# Autodesk Inventor assembly: Shade 02 with LEDs 01
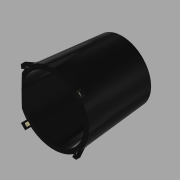
[picture p0: Inventor's stored thumbnail of the model, 180x180]
Saved by Autodesk Inventor 2020 (Build 240168000, 168)
## iProperties
Created: 2019-07-25
Part Number: Shade 02 with LEDs 01
Document SubType Name: Assembly
Designer: Ben
Author: Ben
## Documents named in this file (3)
- C:\Users\Ben\Documents\Inventor\HydraVivarium\Shade 02 with LEDs 01.iam
- C:\Users\Ben\Documents\Inventor\HydraVivarium\Lens Shade and Light 02.ipt
- C:\Users\Ben\Documents\Inventor\HydraVivarium\SFH4451 Narrow Beam IR LED.ipt
## Components (5 placed, 2 different names)
1. Lens Shade and Light 02:1 — Mate:1, Mate:2, Mate:3
2. SFH4451 Narrow Beam IR LED:1 — Mate:1, Mate:2, Mate:3
3. SFH4451 Narrow Beam IR LED:2
4. SFH4451 Narrow Beam IR LED:3
5. SFH4451 Narrow Beam IR LED:4
## Component patterns: (4 elements, first: SFH4451 Narrow Beam IR LED:1)
## Relationships (3: Mate 3)
- Mate:1: Lens Shade and Light 02:1 ↔ SFH4451 Narrow Beam IR LED:1
- Mate:2: Lens Shade and Light 02:1 ↔ SFH4451 Narrow Beam IR LED:1
- Mate:3 (0.2 mm): Lens Shade and Light 02:1 ↔ SFH4451 Narrow Beam IR LED:1
